# Autodesk Inventor assembly: Ensamble_Final
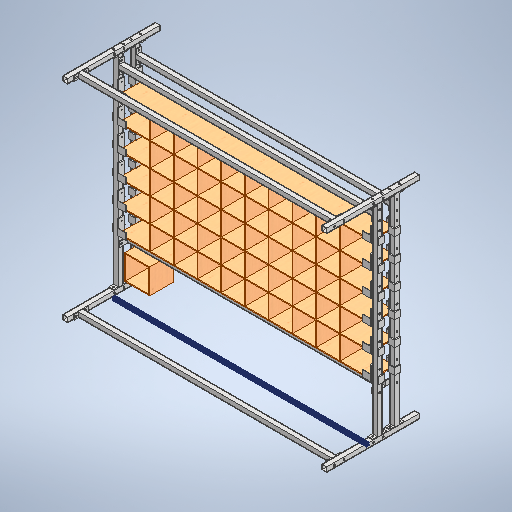
[picture p0: Inventor's stored thumbnail of the model, 512x512]
Saved by Autodesk Inventor 2025.2 (Build 292293000, 293)
## iProperties
Created: 2025-05-30
Part Number: Ensamble_Final
Document SubType Name: Assembly
Designer: USER
Author: USER
## Documents named in this file (10)
- C:\Users\USER\Desktop\TESIS\STORAGE_FINAL\Ensamble_Final.iam
- C:\Users\USER\Desktop\TESIS\STORAGE_FINAL\Perfil_Vertical_Acero.ipt
- C:\Users\USER\Desktop\TESIS\STORAGE_FINAL\Sujetadores.ipt
- C:\Users\USER\Desktop\TESIS\STORAGE_FINAL\Subensamble estaciones.iam
- C:\Users\USER\Desktop\TESIS\STORAGE_FINAL\Sujetador_Mirror.ipt
- C:\Users\USER\Desktop\TESIS\STORAGE_FINAL\Base_Fija_Acero.ipt
- C:\Users\USER\Desktop\TESIS\STORAGE_FINAL\Bases_Perfiles_Acero.ipt
- C:\Users\USER\Desktop\TESIS\STORAGE_FINAL\Estacion.ipt
- C:\Users\USER\Desktop\TESIS\STORAGE_FINAL\Bases_MDF_Acero.ipt
- C:\Users\USER\Desktop\TESIS\STORAGE_FINAL\Aluminio estructural 20x 20_ eje x.ipt
## Components (40 placed, 9 different names)
1. Perfil_Vertical_Acero:1 — Mate:1, Mate:2, Mate:3, Mate:4, Mate:5, Mate:6, Mate:7, Mate:8, Mate:9, Mate:10, Mate:11, Mate:12, Mate:13, Mate:14, Mate:15, Mate:16, Mate:17, Mate:18, Mate:86, Mate:88, Mate:101, Mate:102, Mate:103, Mate:114, Mate:115, Mate:125
2. Sujetadores:2 — Mate:1, Mate:2, Mate:3, Mate:19, Mate:20, Mate:21
3. Sujetadores:3 — Mate:4, Mate:5, Mate:6
4. Sujetadores:4 — Mate:7, Mate:8, Mate:9
5. Sujetadores:5 — Mate:10, Mate:11, Mate:12
6. Sujetadores:6 — Mate:13, Mate:14, Mate:15
7. Sujetadores:7 — Mate:16, Mate:17, Mate:18
8. Subensamble estaciones:1 [sub-assembly] — Mate:19, Mate:20, Mate:21, Mate:41, Mate:42, Mate:43, Mate:59, Mate:60, Mate:61, Mate:83, Mate:84, Mate:85, Flush:1, Flush:2
9. Perfil_Vertical_Acero:2 — Mate:23, Mate:24, Mate:25, Mate:26, Mate:27, Mate:28, Mate:29, Mate:30, Mate:31, Mate:32, Mate:33, Mate:34, Mate:35, Mate:36, Mate:37, Mate:38, Mate:39, Mate:40, Mate:91, Mate:92, Mate:93, Mate:94, Mate:95, Mate:121, Mate:122, Mate:123
10. Sujetadores:8 — Mate:23, Mate:24, Mate:25, Mate:41, Mate:42, Mate:43
11. Sujetadores:9 — Mate:26, Mate:27, Mate:28
12. Sujetadores:10 — Mate:29, Mate:30, Mate:31
13. Sujetadores:11 — Mate:32, Mate:33, Mate:34
14. Sujetadores:12 — Mate:35, Mate:36, Mate:37
15. Sujetadores:13 — Mate:38, Mate:39, Mate:40
16. Sujetador_Mirror:2 — Mate:44, Mate:45, Mate:46, Mate:59, Mate:60, Mate:61
17. Sujetador_Mirror:3 — Mate:47, Mate:48, Mate:49
18. Sujetador_Mirror:4 — Mate:53, Mate:54, Mate:55
19. Sujetador_Mirror:5 — Mate:56, Mate:57, Mate:58
20. Sujetador_Mirror:6 — Mate:50, Mate:51, Mate:52
21. Perfil_Vertical_Acero:3 — Mate:44, Mate:45, Mate:46, Mate:47, Mate:48, Mate:49, Mate:50, Mate:51, Mate:52, Mate:53, Mate:54, Mate:55, Mate:56, Mate:57, Mate:58, Mate:62, Mate:63, Mate:64, Mate:89, Mate:90, Mate:96, Mate:97, Mate:98, Mate:116, Mate:117, Mate:118
22. Sujetador_Mirror:7 — Mate:62, Mate:63, Mate:64
23. Perfil_Vertical_Acero:4 — Mate:65, Mate:66, Mate:67, Mate:68, Mate:69, Mate:70, Mate:71, Mate:72, Mate:73, Mate:74, Mate:75, Mate:76, Mate:77, Mate:78, Mate:79, Mate:80, Mate:81, Mate:82, Mate:87, Mate:99, Mate:100, Mate:119, Mate:120, Mate:126, Mate:127
24. Sujetador_Mirror:8 — Mate:77, Mate:78, Mate:79
25. Sujetador_Mirror:9 — Mate:74, Mate:75, Mate:76
26. Sujetador_Mirror:10 — Mate:68, Mate:69, Mate:70
27. Sujetador_Mirror:11 — Mate:65, Mate:66, Mate:67
28. Sujetador_Mirror:12 — Mate:80, Mate:81, Mate:82, Mate:83, Mate:84, Mate:85
29. Sujetador_Mirror:13 — Mate:71, Mate:72, Mate:73
30. Base_Fija_Acero:1 — Mate:86, Mate:87, Mate:88, Mate:109, Mate:110
31. Base_Fija_Acero:2 — Mate:89, Mate:90, Mate:91, Mate:92, Mate:93, Mate:111, Mate:112, Mate:113
32. Base_Fija_Acero:3 — Mate:99, Mate:100, Mate:101, Mate:102, Mate:103, Mate:104, Mate:105
33. Base_Fija_Acero:4 — Mate:94, Mate:95, Mate:96, Mate:97, Mate:98, Mate:106, Mate:107, Mate:108
34. Bases_Perfiles_Acero:1 — Mate:104, Mate:105, Mate:106, Mate:107, Mate:108
35. Bases_Perfiles_Acero:2 — Mate:109, Mate:110, Mate:111, Mate:112, Mate:113
36. Bases_Perfiles_Acero:3 — Mate:114, Mate:115, Mate:116, Mate:117, Mate:118
37. Bases_Perfiles_Acero:4 — Mate:119, Mate:120, Mate:121, Mate:122, Mate:123
38. Estacion:1 — Flush:1, Flush:2, Mate:128
39. Bases_MDF_Acero:1 — Mate:125, Mate:126, Mate:127, Mate:128
40. Aluminio estructural 20x 20_ eje x:1
## Relationships (128: Mate 126, Flush 2)
- Mate:1: Perfil_Vertical_Acero:1 ↔ Sujetadores:2
- Mate:2: Perfil_Vertical_Acero:1 ↔ Sujetadores:2
- Mate:3: Perfil_Vertical_Acero:1 ↔ Sujetadores:2
- Mate:4: Perfil_Vertical_Acero:1 ↔ Sujetadores:3
- Mate:5: Perfil_Vertical_Acero:1 ↔ Sujetadores:3
- Mate:6: Perfil_Vertical_Acero:1 ↔ Sujetadores:3
- Mate:7: Perfil_Vertical_Acero:1 ↔ Sujetadores:4
- Mate:8: Perfil_Vertical_Acero:1 ↔ Sujetadores:4
- Mate:9: Perfil_Vertical_Acero:1 ↔ Sujetadores:4
- Mate:10: Perfil_Vertical_Acero:1 ↔ Sujetadores:5
- Mate:11: Perfil_Vertical_Acero:1 ↔ Sujetadores:5
- Mate:12: Perfil_Vertical_Acero:1 ↔ Sujetadores:5
- Mate:13: Perfil_Vertical_Acero:1 ↔ Sujetadores:6
- Mate:14: Perfil_Vertical_Acero:1 ↔ Sujetadores:6
- Mate:15: Perfil_Vertical_Acero:1 ↔ Sujetadores:6
- Mate:16: Perfil_Vertical_Acero:1 ↔ Sujetadores:7
- Mate:17: Perfil_Vertical_Acero:1 ↔ Sujetadores:7
- Mate:18: Perfil_Vertical_Acero:1 ↔ Sujetadores:7
- Mate:19: Sujetadores:2 ↔ Subensamble estaciones:1
- Mate:20: Sujetadores:2 ↔ Subensamble estaciones:1
- Mate:21: Sujetadores:2 ↔ Subensamble estaciones:1
- Mate:23: Perfil_Vertical_Acero:2 ↔ Sujetadores:8
- Mate:24: Perfil_Vertical_Acero:2 ↔ Sujetadores:8
- Mate:25: Perfil_Vertical_Acero:2 ↔ Sujetadores:8
- Mate:26: Perfil_Vertical_Acero:2 ↔ Sujetadores:9
- Mate:27: Perfil_Vertical_Acero:2 ↔ Sujetadores:9
- Mate:28: Perfil_Vertical_Acero:2 ↔ Sujetadores:9
- Mate:29: Perfil_Vertical_Acero:2 ↔ Sujetadores:10
- Mate:30: Perfil_Vertical_Acero:2 ↔ Sujetadores:10
- Mate:31: Perfil_Vertical_Acero:2 ↔ Sujetadores:10
- Mate:32: Perfil_Vertical_Acero:2 ↔ Sujetadores:11
- Mate:33: Perfil_Vertical_Acero:2 ↔ Sujetadores:11
- Mate:34: Perfil_Vertical_Acero:2 ↔ Sujetadores:11
- Mate:35: Perfil_Vertical_Acero:2 ↔ Sujetadores:12
- Mate:36: Perfil_Vertical_Acero:2 ↔ Sujetadores:12
- Mate:37: Perfil_Vertical_Acero:2 ↔ Sujetadores:12
- Mate:38: Perfil_Vertical_Acero:2 ↔ Sujetadores:13
- Mate:39: Perfil_Vertical_Acero:2 ↔ Sujetadores:13
- Mate:40: Perfil_Vertical_Acero:2 ↔ Sujetadores:13
- Mate:41: Subensamble estaciones:1 ↔ Sujetadores:8
- Mate:42: Subensamble estaciones:1 ↔ Sujetadores:8
- Mate:43: Subensamble estaciones:1 ↔ Sujetadores:8
- Mate:44: Sujetador_Mirror:2 ↔ Perfil_Vertical_Acero:3
- Mate:45: Sujetador_Mirror:2 ↔ Perfil_Vertical_Acero:3
- Mate:46: Sujetador_Mirror:2 ↔ Perfil_Vertical_Acero:3
- Mate:47: Sujetador_Mirror:3 ↔ Perfil_Vertical_Acero:3
- Mate:48: Sujetador_Mirror:3 ↔ Perfil_Vertical_Acero:3
- Mate:49: Sujetador_Mirror:3 ↔ Perfil_Vertical_Acero:3
- Mate:50: Sujetador_Mirror:6 ↔ Perfil_Vertical_Acero:3
- Mate:51: Sujetador_Mirror:6 ↔ Perfil_Vertical_Acero:3
- Mate:52: Sujetador_Mirror:6 ↔ Perfil_Vertical_Acero:3
- Mate:53: Sujetador_Mirror:4 ↔ Perfil_Vertical_Acero:3
- Mate:54: Sujetador_Mirror:4 ↔ Perfil_Vertical_Acero:3
- Mate:55: Sujetador_Mirror:4 ↔ Perfil_Vertical_Acero:3
- Mate:56: Sujetador_Mirror:5 ↔ Perfil_Vertical_Acero:3
- Mate:57: Sujetador_Mirror:5 ↔ Perfil_Vertical_Acero:3
- Mate:58: Sujetador_Mirror:5 ↔ Perfil_Vertical_Acero:3
- Mate:59: Subensamble estaciones:1 ↔ Sujetador_Mirror:2
- Mate:60: Subensamble estaciones:1 ↔ Sujetador_Mirror:2
- Mate:61: Subensamble estaciones:1 ↔ Sujetador_Mirror:2
- Mate:62: Perfil_Vertical_Acero:3 ↔ Sujetador_Mirror:7
- Mate:63: Perfil_Vertical_Acero:3 ↔ Sujetador_Mirror:7
- Mate:64: Perfil_Vertical_Acero:3 ↔ Sujetador_Mirror:7
- Mate:65: Perfil_Vertical_Acero:4 ↔ Sujetador_Mirror:11
- Mate:66: Perfil_Vertical_Acero:4 ↔ Sujetador_Mirror:11
- Mate:67: Perfil_Vertical_Acero:4 ↔ Sujetador_Mirror:11
- Mate:68: Perfil_Vertical_Acero:4 ↔ Sujetador_Mirror:10
- Mate:69: Perfil_Vertical_Acero:4 ↔ Sujetador_Mirror:10
- Mate:70: Perfil_Vertical_Acero:4 ↔ Sujetador_Mirror:10
- Mate:71: Perfil_Vertical_Acero:4 ↔ Sujetador_Mirror:13
- Mate:72: Perfil_Vertical_Acero:4 ↔ Sujetador_Mirror:13
- Mate:73: Perfil_Vertical_Acero:4 ↔ Sujetador_Mirror:13
- Mate:74: Perfil_Vertical_Acero:4 ↔ Sujetador_Mirror:9
- Mate:75: Perfil_Vertical_Acero:4 ↔ Sujetador_Mirror:9
- Mate:76: Perfil_Vertical_Acero:4 ↔ Sujetador_Mirror:9
- Mate:77: Perfil_Vertical_Acero:4 ↔ Sujetador_Mirror:8
- Mate:78: Perfil_Vertical_Acero:4 ↔ Sujetador_Mirror:8
- Mate:79: Perfil_Vertical_Acero:4 ↔ Sujetador_Mirror:8
- Mate:80: Perfil_Vertical_Acero:4 ↔ Sujetador_Mirror:12
- Mate:81: Perfil_Vertical_Acero:4 ↔ Sujetador_Mirror:12
- Mate:82: Perfil_Vertical_Acero:4 ↔ Sujetador_Mirror:12
- Mate:83: Subensamble estaciones:1 ↔ Sujetador_Mirror:12
- Mate:84: Subensamble estaciones:1 ↔ Sujetador_Mirror:12
- Mate:85: Subensamble estaciones:1 ↔ Sujetador_Mirror:12
- Mate:86: Perfil_Vertical_Acero:1 ↔ Base_Fija_Acero:1
- Mate:87: Perfil_Vertical_Acero:4 ↔ Base_Fija_Acero:1
- Mate:88: Perfil_Vertical_Acero:1 ↔ Base_Fija_Acero:1
- Mate:89: Perfil_Vertical_Acero:3 ↔ Base_Fija_Acero:2
- Mate:90: Perfil_Vertical_Acero:3 ↔ Base_Fija_Acero:2
- Mate:91: Perfil_Vertical_Acero:2 ↔ Base_Fija_Acero:2
- Mate:92: Perfil_Vertical_Acero:2 ↔ Base_Fija_Acero:2
- Mate:93: Perfil_Vertical_Acero:2 ↔ Base_Fija_Acero:2
- Mate:94: Perfil_Vertical_Acero:2 ↔ Base_Fija_Acero:4
- Mate:95: Perfil_Vertical_Acero:2 ↔ Base_Fija_Acero:4
- Mate:96: Perfil_Vertical_Acero:3 ↔ Base_Fija_Acero:4
- Mate:97: Perfil_Vertical_Acero:3 ↔ Base_Fija_Acero:4
- Mate:98: Perfil_Vertical_Acero:3 ↔ Base_Fija_Acero:4
- Mate:99: Perfil_Vertical_Acero:4 ↔ Base_Fija_Acero:3
- Mate:100: Perfil_Vertical_Acero:4 ↔ Base_Fija_Acero:3
- Mate:101: Perfil_Vertical_Acero:1 ↔ Base_Fija_Acero:3
- Mate:102: Perfil_Vertical_Acero:1 ↔ Base_Fija_Acero:3
- Mate:103: Perfil_Vertical_Acero:1 ↔ Base_Fija_Acero:3
- Mate:104: Base_Fija_Acero:3 ↔ Bases_Perfiles_Acero:1
- Mate:105: Base_Fija_Acero:3 ↔ Bases_Perfiles_Acero:1
- Mate:106: Base_Fija_Acero:4 ↔ Bases_Perfiles_Acero:1
- Mate:107: Base_Fija_Acero:4 ↔ Bases_Perfiles_Acero:1
- Mate:108: Base_Fija_Acero:4 ↔ Bases_Perfiles_Acero:1
- Mate:109: Base_Fija_Acero:1 ↔ Bases_Perfiles_Acero:2
- Mate:110: Base_Fija_Acero:1 ↔ Bases_Perfiles_Acero:2
- Mate:111: Base_Fija_Acero:2 ↔ Bases_Perfiles_Acero:2
- Mate:112: Base_Fija_Acero:2 ↔ Bases_Perfiles_Acero:2
- Mate:113: Base_Fija_Acero:2 ↔ Bases_Perfiles_Acero:2
- Mate:114: Perfil_Vertical_Acero:1 ↔ Bases_Perfiles_Acero:3
- Mate:115: Perfil_Vertical_Acero:1 ↔ Bases_Perfiles_Acero:3
- Mate:116: Perfil_Vertical_Acero:3 ↔ Bases_Perfiles_Acero:3
- Mate:117: Perfil_Vertical_Acero:3 ↔ Bases_Perfiles_Acero:3
- Mate:118: Perfil_Vertical_Acero:3 ↔ Bases_Perfiles_Acero:3
- Mate:119: Perfil_Vertical_Acero:4 ↔ Bases_Perfiles_Acero:4
- Mate:120: Perfil_Vertical_Acero:4 ↔ Bases_Perfiles_Acero:4
- Mate:121: Perfil_Vertical_Acero:2 ↔ Bases_Perfiles_Acero:4
- Mate:122: Perfil_Vertical_Acero:2 ↔ Bases_Perfiles_Acero:4
- Mate:123: Perfil_Vertical_Acero:2 ↔ Bases_Perfiles_Acero:4
- Flush:1: Subensamble estaciones:1 ↔ Estacion:1
- Flush:2: Subensamble estaciones:1 ↔ Estacion:1
- Mate:125: Perfil_Vertical_Acero:1 ↔ Bases_MDF_Acero:1
- Mate:126: Perfil_Vertical_Acero:4 ↔ Bases_MDF_Acero:1
- Mate:127: Perfil_Vertical_Acero:4 ↔ Bases_MDF_Acero:1
- Mate:128: Estacion:1 ↔ Bases_MDF_Acero:1
